# Autodesk Inventor assembly: 6 bar_MIR
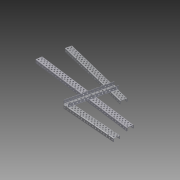
[picture p0: Inventor's stored thumbnail of the model, 180x180]
Saved by Autodesk Inventor 2014 SP1 (Build 180222100, 222)
## iProperties
Created: 2014-02-27
Part Number: 6 bar_MIR
Document SubType Name: Assembly
Designer: Ryan
Author: Ryan
## Documents named in this file (10)
- C:\Users\Ryan\Desktop\sw\toss up 4th robot\6 bar\6 bar_MIR.iam
- C:\Users\Ryan\Desktop\sw\lib\Aperture VEX CAD Library\Metal\C Channel\2 x 25.ipt
- C:\Users\Ryan\Desktop\sw\lib\Aperture VEX CAD Library\Metal\C Channel\2 x 35.ipt
- C:\Users\Ryan\Desktop\sw\lib\Aperture VEX CAD Library\Spacers\thin\SPACER-0320-00625.ipt
- C:\Users\Ryan\Desktop\sw\lib\Aperture VEX CAD Library\Bearing Blocks\Bearing Block.ipt
- C:\Users\Ryan\Desktop\sw\lib\Aperture VEX CAD Library\Metal\C Channel\2 x 17.ipt
- C:\Users\Ryan\Desktop\sw\lib\Aperture VEX CAD Library\Hardware\8-32\Shoulder Screw_MIR.ipt
- C:\Users\Ryan\Desktop\sw\lib\Aperture VEX CAD Library\Hardware\8-32\Shoulder Screw.ipt
- C:\Users\Ryan\Desktop\sw\lib\Aperture VEX CAD Library\Metal\C Channel\2 x 14.ipt
- C:\Users\Ryan\Desktop\sw\lib\Aperture VEX CAD Library\Hardware\8-32\8-32 nylock.ipt
## Components (17 placed, 9 different names)
1. 2 x 25:1 — Mate:25, Mate:24, Mate:23, Mate:32, Mate:31, Mate:30, Mate:37, Mate:42, Mate:46
2. 2 x 35:1 — Mate:19, Mate:18, Mate:10, Mate:14, Mate:13, Mate:12, Mate:11, Mate:28, Mate:27, Mate:26, Mate:34, Mate:43
3. SPACER-0320-00625:1 — Mate:17, Mate:16, Mate:15, Mate:38, Mate:48
4. SPACER-0320-00625:2 — Mate:19, Mate:18, Mate:10, Mate:35, Mate:40
5. Bearing Block:1 — Mate:14, Mate:13, Mate:12, Mate:11
6. 2 x 17:1 — Mate:17, Mate:16, Mate:15, Mate:39, Mate:51, Mate:50, Mate:49, Mate:41
7. SPACER-0320-00625:3 — Mate:25, Mate:24, Mate:23, Mate:36, Mate:47, Mate:46
8. Bearing Block:2 — Mate:28, Mate:27, Mate:26, Mate:43
9. Bearing Block:3 — Mate:32, Mate:31, Mate:30, Mate:42
10. Shoulder Screw_MIR:1 — Mate:35, Mate:34, Mate:44, Mate:43, Mate:44, Mate:45, Mate:49
11. Shoulder Screw:1 — Mate:37, Mate:36, Mate:42, Mate:41, Mate:51
12. Shoulder Screw:2 — Mate:39, Mate:38, Mate:46, Mate:45, Mate:47
13. 2 x 14:1 — Mate:48, Mate:47, Mate:46, Mate:45, Mate:44, Mate:43, Mate:42, Mate:41, Mate:40, Mate:44, Mate:45, Mate:48, Mate:50, Mate:52
14. Bearing Block:4 — Mate:51, Mate:50, Mate:49, Mate:41
15. 8-32 nylock:1 — Mate:47, Mate:48
16. 8-32 nylock:2 — Mate:49, Mate:50
17. 8-32 nylock:3 — Mate:51, Mate:52
## Relationships (49: Mate 49)
- Mate:19 (-10.3886 mm): 2 x 35:1 ↔ SPACER-0320-00625:2
- Mate:18 (2.3114 mm): 2 x 35:1 ↔ SPACER-0320-00625:2
- Mate:10: 2 x 35:1 ↔ SPACER-0320-00625:2
- Mate:14 (2.3114 mm): 2 x 35:1 ↔ Bearing Block:1
- Mate:13 (2.3114 mm): 2 x 35:1 ↔ Bearing Block:1
- Mate:12 (2.3114 mm): 2 x 35:1 ↔ Bearing Block:1
- Mate:11: 2 x 35:1 ↔ Bearing Block:1
- Mate:17 (2.3114 mm): SPACER-0320-00625:1 ↔ 2 x 17:1
- Mate:16 (2.3114 mm): SPACER-0320-00625:1 ↔ 2 x 17:1
- Mate:15: SPACER-0320-00625:1 ↔ 2 x 17:1
- Mate:25 (2.3114 mm): 2 x 25:1 ↔ SPACER-0320-00625:3
- Mate:24 (-2.3114 mm): 2 x 25:1 ↔ SPACER-0320-00625:3
- Mate:23: 2 x 25:1 ↔ SPACER-0320-00625:3
- Mate:28: 2 x 35:1 ↔ Bearing Block:2
- Mate:27 (2.3114 mm): 2 x 35:1 ↔ Bearing Block:2
- Mate:26 (2.3114 mm): 2 x 35:1 ↔ Bearing Block:2
- Mate:32 (2.3114 mm): 2 x 25:1 ↔ Bearing Block:3
- Mate:31 (2.3114 mm): 2 x 25:1 ↔ Bearing Block:3
- Mate:30: 2 x 25:1 ↔ Bearing Block:3
- Mate:35: SPACER-0320-00625:2 ↔ Shoulder Screw_MIR:1
- Mate:34: 2 x 35:1 ↔ Shoulder Screw_MIR:1
- Mate:37: 2 x 25:1 ↔ Shoulder Screw:1
- Mate:36: SPACER-0320-00625:3 ↔ Shoulder Screw:1
- Mate:39: 2 x 17:1 ↔ Shoulder Screw:2
- Mate:38: SPACER-0320-00625:1 ↔ Shoulder Screw:2
- Mate:48: SPACER-0320-00625:1 ↔ 2 x 14:1
- Mate:47: SPACER-0320-00625:3 ↔ 2 x 14:1
- Mate:46 (2.3114 mm): Shoulder Screw:2 ↔ 2 x 14:1
- Mate:45 (2.3114 mm): Shoulder Screw:2 ↔ 2 x 14:1
- Mate:44 (2.3114 mm): Shoulder Screw_MIR:1 ↔ 2 x 14:1
- Mate:43 (2.3114 mm): Shoulder Screw_MIR:1 ↔ 2 x 14:1
- Mate:42 (2.3114 mm): Shoulder Screw:1 ↔ 2 x 14:1
- Mate:41 (2.3114 mm): Shoulder Screw:1 ↔ 2 x 14:1
- Mate:40: SPACER-0320-00625:2 ↔ 2 x 14:1
- Mate:51 (2.3114 mm): 2 x 17:1 ↔ Bearing Block:4
- Mate:50 (2.3114 mm): 2 x 17:1 ↔ Bearing Block:4
- Mate:49: 2 x 17:1 ↔ Bearing Block:4
- Mate:41 (2.3114 mm): 2 x 17:1 ↔ Bearing Block:4
- Mate:42 (2.3114 mm): 2 x 25:1 ↔ Bearing Block:3
- Mate:43 (2.3114 mm): 2 x 35:1 ↔ Bearing Block:2
- Mate:44 (2.3114 mm): Shoulder Screw_MIR:1 ↔ 2 x 14:1
- Mate:45 (2.3114 mm): Shoulder Screw_MIR:1 ↔ 2 x 14:1
- Mate:46 (2.3114 mm): 2 x 25:1 ↔ SPACER-0320-00625:3
- Mate:47: Shoulder Screw:2 ↔ 8-32 nylock:1
- Mate:48: 2 x 14:1 ↔ 8-32 nylock:1
- Mate:49: Shoulder Screw_MIR:1 ↔ 8-32 nylock:2
- Mate:50: 2 x 14:1 ↔ 8-32 nylock:2
- Mate:51: Shoulder Screw:1 ↔ 8-32 nylock:3
- Mate:52: 2 x 14:1 ↔ 8-32 nylock:3
## Named parameters: q = 2.3114 mm
